# Autodesk Inventor assembly: X02598_LEGOmini_UpperBody
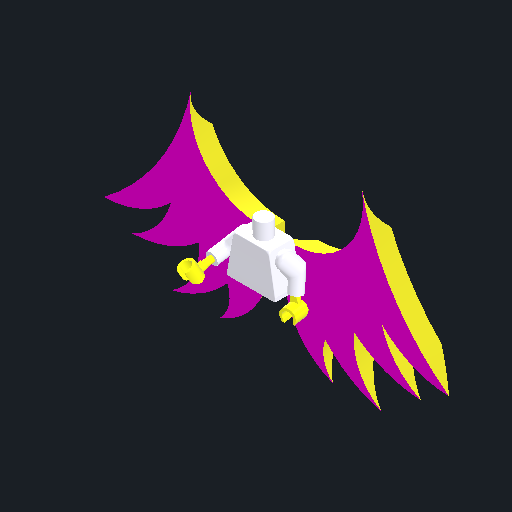
[picture p0: Inventor's stored thumbnail of the model, 512x512]
Saved by Autodesk Inventor 2022 (Build 260153000, 153)
## iProperties
Created: 2022-02-05
Part Number: X02598_LEGOmini_UpperBody
Document SubType Name: Assembly
Designer: Jason
Author: Jason
## Documents named in this file (5)
- D:\D-disk\pomelo\大一\下學期\機械設計製圖\110033226_LEGOmini\110033226_LEGOmini_天使\110033226_LEGOmini_天使上半身.iam
- D:\D-disk\pomelo\大一\下學期\機械設計製圖\110033226_LEGOmini\110033226_LEGOmini_天使\110033226_LEGOmini_天使上半身.ipt
- D:\D-disk\pomelo\大一\下學期\機械設計製圖\110033226_LEGOmini\110033226_LEGOmini_天使\110033226_LEGOmini_左手臂.ipt
- D:\D-disk\pomelo\大一\下學期\機械設計製圖\110033226_LEGOmini\110033226_LEGOmini_天使\110033226_LEGOmini_右手臂.ipt
- D:\D-disk\pomelo\大一\下學期\機械設計製圖\110033226_LEGOmini\110033226_LEGOmini_天使\110033226_LEGOmini_手心.ipt
## Components (5 placed, 4 different names)
1. 110033226_LEGOmini_天使上半身:1 — 插入:1, 插入:2
2. 110033226_LEGOmini_左手臂:1 — 插入:1, 貼合:2
3. 110033226_LEGOmini_右手臂:1 — 插入:2, 貼合:1
4. 110033226_LEGOmini_手心:1 — 貼合:1
5. 110033226_LEGOmini_手心:2 — 貼合:2
## Relationships (4: Insert 2, Mate 2)
- 插入:1 [Insert]: 110033226_LEGOmini_天使上半身:1 ↔ 110033226_LEGOmini_左手臂:1
- 插入:2 [Insert]: 110033226_LEGOmini_天使上半身:1 ↔ 110033226_LEGOmini_右手臂:1
- 貼合:1 [Mate]: 110033226_LEGOmini_右手臂:1 ↔ 110033226_LEGOmini_手心:1
- 貼合:2 [Mate]: 110033226_LEGOmini_左手臂:1 ↔ 110033226_LEGOmini_手心:2
